# Autodesk Inventor assembly: Custom Cover Assembly
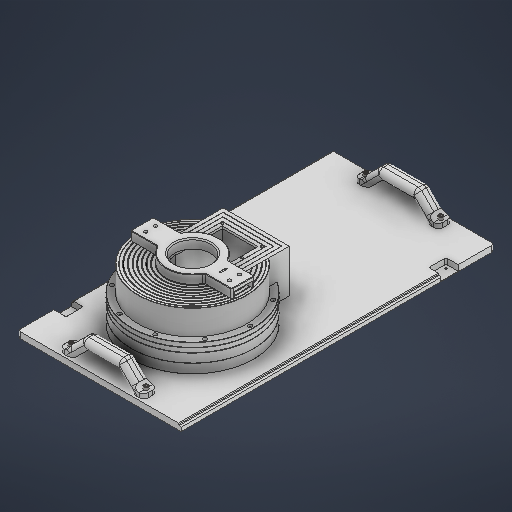
[picture p0: Inventor's stored thumbnail of the model, 512x512]
Saved by Autodesk Inventor 2025 (Build 290162000, 162)
## iProperties
Created: 2024-04-26
Part Number: Custom Cover Assembly
Document SubType Name: Assembly
Designer: Thienan Hoang
Author: Thienan Hoang
## Documents named in this file (15)
- C:\Users\mayhe\OneDrive\Documents\GitHub\In-situ-monitoring-of-powder-bed-fusion-additive-manufacturing\system_development\Orichalcum\v0.2\Hardware_design\custom-cover\Custom Cover Full Assembly v0.2.iam
- C:\Users\mayhe\OneDrive\Documents\GitHub\In-situ-monitoring-of-powder-bed-fusion-additive-manufacturing\system_development\Orichalcum\v0.2\Hardware_design\custom-cover\cover\Updated Cover.ipt
- C:\Users\mayhe\OneDrive\Documents\GitHub\In-situ-monitoring-of-powder-bed-fusion-additive-manufacturing\system_development\Orichalcum\v0.2\Hardware_design\custom-cover\cylinder-parts\final-parts\Cylinder Slidey Bit.iam
- C:\Users\mayhe\OneDrive\Documents\GitHub\In-situ-monitoring-of-powder-bed-fusion-additive-manufacturing\system_development\Orichalcum\v0.2\Hardware_design\custom-cover\cylinder-parts\final-parts\Cylinder Spacer 25mm.ipt
- C:\Users\mayhe\OneDrive\Documents\GitHub\In-situ-monitoring-of-powder-bed-fusion-additive-manufacturing\system_development\Orichalcum\v0.2\Hardware_design\custom-cover\cover\Handles.ipt
- C:\Users\mayhe\OneDrive\Documents\GitHub\In-situ-monitoring-of-powder-bed-fusion-additive-manufacturing\system_development\Orichalcum\v0.2\Hardware_design\custom-cover\8020-parts\ANSI B18.3.1M - M6x1 x 20(1).ipt
- C:\Users\mayhe\OneDrive\Documents\GitHub\In-situ-monitoring-of-powder-bed-fusion-additive-manufacturing\system_development\Orichalcum\v0.2\Hardware_design\custom-cover\cylinder-parts\final-parts\Cylinder Bottom Ring.ipt
- C:\Users\mayhe\OneDrive\Documents\GitHub\In-situ-monitoring-of-powder-bed-fusion-additive-manufacturing\system_development\Orichalcum\v0.2\Hardware_design\custom-cover\cylinder-parts\Galvo Housing\Galvo Housing 1\Galvo Housing-01.ipt
- C:\Users\mayhe\OneDrive\Documents\GitHub\In-situ-monitoring-of-powder-bed-fusion-additive-manufacturing\system_development\Orichalcum\v0.2\Hardware_design\custom-cover\cylinder-parts\Galvo Housing\Galvo Housing 1.ipt
- C:\Users\mayhe\OneDrive\Documents\GitHub\In-situ-monitoring-of-powder-bed-fusion-additive-manufacturing\system_development\Orichalcum\v0.2\Hardware_design\custom-cover\cylinder-parts\Galvo Housing\Galvo Housing 2\Galvo Housing-01.ipt
- C:\Users\mayhe\OneDrive\Documents\GitHub\In-situ-monitoring-of-powder-bed-fusion-additive-manufacturing\system_development\Orichalcum\v0.2\Hardware_design\custom-cover\cylinder-parts\Galvo Housing\Galvo Housing 2.ipt
- C:\Users\mayhe\OneDrive\Documents\GitHub\In-situ-monitoring-of-powder-bed-fusion-additive-manufacturing\system_development\Orichalcum\v0.2\Hardware_design\custom-cover\cylinder-parts\Galvo Housing\Galvo Housing 3\Galvo Housing-01.ipt
- C:\Users\mayhe\OneDrive\Documents\GitHub\In-situ-monitoring-of-powder-bed-fusion-additive-manufacturing\system_development\Orichalcum\v0.2\Hardware_design\custom-cover\cylinder-parts\Galvo Housing\Galvo Housing 3.ipt
- C:\Users\mayhe\OneDrive\Documents\GitHub\In-situ-monitoring-of-powder-bed-fusion-additive-manufacturing\system_development\Orichalcum\v0.2\Hardware_design\custom-cover\cylinder-parts\Galvo Housing\Galvo Housing 4\Galvo Housing-01.ipt
- C:\Users\mayhe\OneDrive\Documents\GitHub\In-situ-monitoring-of-powder-bed-fusion-additive-manufacturing\system_development\Orichalcum\v0.2\Hardware_design\custom-cover\cylinder-parts\Galvo Housing\Galvo Housing 4.ipt
## Components (14 placed, 7 different names)
1. Updated Cover:1 — Flush:5, Mate:48, Mate:106, Mate:107, Mate:108, Mate:109, Mate:110
2. Cylinder Spacer 25mm:1 — Rotational:3
3. Cylinder Slidey Bit:1 [sub-assembly] — Rotational:3, Mate:111, Mate:112, Mate:114, Mate:118, Mate:120
4. Handles:1 — Mate:108, Mate:109, Insert:18, Insert:19
5. Handles:2 — Mate:106, Mate:107, Insert:20, Insert:21
6. Cylinder Bottom Ring:1 — Mate:110, Mate:113
7. Galvo Housing-01:1 — Mate:111, Mate:112, Mate:113, Mate:115, Mate:116, Mate:117, Mate:122
8. Galvo Housing-01:1 — Mate:114, Mate:115, Mate:116, Mate:119
9. Galvo Housing-01:1 — Mate:117, Mate:118, Mate:119, Mate:121
10. Galvo Housing-01:1 — Mate:120, Mate:121, Mate:122
11. Forged Socket Head Cap Screw - Metric M6x1 x 20:1 — Insert:18
12. Forged Socket Head Cap Screw - Metric M6x1 x 20:2 — Insert:19
13. Forged Socket Head Cap Screw - Metric M6x1 x 20:3 — Insert:20
14. Forged Socket Head Cap Screw - Metric M6x1 x 20:4 — Insert:21
## Relationships (25: Mate 18, Insert 4, Flush 2, RevoluteJoint 1)
- Flush:5 (180 mm): Updated Cover:1
- Mate:48: Updated Cover:1
- Flush:6 (38 mm)
- Mate:106: Updated Cover:1 ↔ Handles:2
- Mate:107: Updated Cover:1 ↔ Handles:2
- Mate:108: Updated Cover:1 ↔ Handles:1
- Mate:109: Updated Cover:1 ↔ Handles:1
- Insert:18: Handles:1 ↔ Forged Socket Head Cap Screw - Metric M6x1 x 20:1
- Insert:19: Handles:1 ↔ Forged Socket Head Cap Screw - Metric M6x1 x 20:2
- Insert:20: Handles:2 ↔ Forged Socket Head Cap Screw - Metric M6x1 x 20:3
- Insert:21: Handles:2 ↔ Forged Socket Head Cap Screw - Metric M6x1 x 20:4
- Rotational:3 [RevoluteJoint]: Cylinder Spacer 25mm:1 ↔ Cylinder Slidey Bit:1
- Mate:110: Updated Cover:1 ↔ Cylinder Bottom Ring:1
- Mate:111: Cylinder Slidey Bit:1 ↔ Galvo Housing-01:1
- Mate:112: Cylinder Slidey Bit:1 ↔ Galvo Housing-01:1
- Mate:113: Cylinder Bottom Ring:1 ↔ Galvo Housing-01:1
- Mate:114: Cylinder Slidey Bit:1 ↔ Galvo Housing-01:1
- Mate:115 (0.5 mm): Galvo Housing-01:1
- Mate:116: Galvo Housing-01:1
- Mate:117: Galvo Housing-01:1
- Mate:118: Cylinder Slidey Bit:1 ↔ Galvo Housing-01:1
- Mate:119 (0.5 mm): Galvo Housing-01:1
- Mate:120: Cylinder Slidey Bit:1 ↔ Galvo Housing-01:1
- Mate:121 (0.5 mm): Galvo Housing-01:1
- Mate:122: Galvo Housing-01:1
